# Autodesk Inventor assembly: NX3224T024_011_Ass
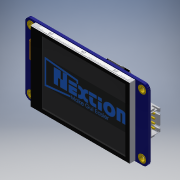
[picture p0: Inventor's stored thumbnail of the model, 180x180]
Saved by Autodesk Inventor 2017 SP1 (Build 210196100, 196)
## iProperties
Created: 2016-08-28
Part Number: NX3224T024_011_Ass
Document SubType Name: Assembly
Designer: jwrjc
Author: jwrjc
## Documents named in this file (14)
- D:\My Projects\Inventor\ElectricalComponents\Nextion_NX3224T024_011\NX3224T024_011_Ass.iam
- D:\My Projects\Inventor\ElectricalComponents\Nextion_NX3224T024_011\NX3224T024_011_PCB.ipt
- D:\My Projects\Inventor\ElectricalComponents\Nextion_NX3224T024_011\AMS1117.ipt
- D:\Documents\Inventor\Content Center Files\R2017\en-US\603_SMD\603_Cap-Lead.ipt
- D:\Documents\Inventor\Content Center Files\R2017\en-US\1206_SMD\1206_Cap.ipt
- D:\My Projects\Inventor\ElectricalComponents\Nextion_NX3224T024_011\603_Resistor.ipt
- D:\My Projects\Inventor\ElectricalComponents\Nextion_NX3224T024_011\IcNextion.ipt
- D:\My Projects\Inventor\ElectricalComponents\Nextion_NX3224T024_011\24_pin_IC.ipt
- D:\My Projects\Inventor\ElectricalComponents\Nextion_NX3224T024_011\16_pin_IC.ipt
- D:\My Projects\Inventor\ElectricalComponents\Nextion_NX3224T024_011\SMD_Trans.ipt
- D:\My Projects\Inventor\ElectricalComponents\Nextion_NX3224T024_011\Micro_SD_Slot.ipt
- D:\My Projects\Inventor\ElectricalComponents\Nextion_NX3224T024_011\SD_Center.ipt
- D:\My Projects\Inventor\ElectricalComponents\Nextion_NX3224T024_011\Nextion_Plug.ipt
- D:\My Projects\Inventor\ElectricalComponents\Nextion_NX3224T024_011\LCD.ipt
## Components (30 placed, 13 different names)
1. NX3224T024_011_PCB:1 — Mate:1, Flush:1, Flush:2, Mate:2, Mate:3, Mate:4, Mate:5, Mate:6, Mate:7, Mate:8, Flush:3, Flush:4, Flush:5, Flush:6, Flush:7, Flush:8, Flush:9, Flush:10, Flush:11, Flush:12, Flush:13, Flush:14, Flush:15, Flush:16, Mate:9, Mate:10, Mate:11, Mate:12, Mate:13, Mate:14, Mate:15, Mate:16, Mate:17, Mate:18, Mate:19, Mate:20, Mate:21, Flush:28, Flush:30, Flush:35, Flush:36, Flush:39, Flush:40, Flush:43, Flush:45, Flush:46, Flush:47, Flush:48, Mate:22, Flush:49, Flush:50
2. AMS1117:1 — Mate:1, Flush:1, Flush:2
3. 603_SMD 603_Cap-Lead:1 — Mate:2, Flush:9, Flush:11
4. 603_SMD 603_Cap-Lead:2 — Mate:3, Flush:8, Flush:10, Flush:37, Flush:38
5. 603_SMD 603_Cap-Lead:3 — Mate:4, Flush:7, Flush:15
6. 603_SMD 603_Cap-Lead:4 — Mate:5, Flush:6, Flush:14, Flush:17, Flush:22
7. 603_SMD 603_Cap-Lead:5 — Mate:6, Flush:5, Flush:12
8. 603_SMD 603_Cap-Lead:6 — Mate:7, Flush:4, Flush:13, Flush:41, Flush:42
9. 1206_SMD 1206_Cap:1 — Mate:8, Flush:3, Flush:16
10. 603_Resistor:1 — Mate:9, Flush:17, Flush:18, Flush:22, Flush:23
11. 603_Resistor:2 — Mate:10, Flush:19, Flush:20, Flush:24, Flush:25
12. 603_Resistor:3 — Mate:11, Flush:21, Flush:26
13. 603_Resistor:4 — Mate:12, Flush:18, Flush:19, Flush:23, Flush:24
14. 603_Resistor:5 — Mate:13, Flush:20, Flush:21, Flush:25, Flush:26
15. 603_Resistor:6 — Mate:14, Flush:27, Flush:29, Flush:36
16. 603_Resistor:7 — Mate:15, Flush:27, Flush:28, Flush:29
17. 603_Resistor:8 — Mate:16, Flush:30, Flush:31, Flush:33
18. 603_Resistor:9 — Mate:17, Flush:31, Flush:32, Flush:33, Flush:34
19. 603_Resistor:10 — Mate:18, Flush:32, Flush:34, Flush:35
20. 603_Resistor:11 — Mate:19, Flush:37, Flush:38
21. 603_Resistor:12 — Mate:20, Flush:41, Flush:42
22. 603_Resistor:13 — Mate:21, Flush:39, Flush:40
23. IcNextion:1
24. 24_pin_IC:1
25. 16_pin_IC:1
26. SMD_Trans:1
27. Micro_SD_Slot:1 — Flush:44, Flush:45
28. SD_Center:1 — Flush:46, Flush:47
29. Nextion_Plug:1 — Flush:48
30. LCD:1 — Mate:22, Flush:49, Flush:50
## Relationships (72: Flush 50, Mate 22)
- Mate:1: NX3224T024_011_PCB:1 ↔ AMS1117:1
- Flush:1 (6 mm): NX3224T024_011_PCB:1 ↔ AMS1117:1
- Flush:2 (12.011 mm): NX3224T024_011_PCB:1 ↔ AMS1117:1
- Mate:2: NX3224T024_011_PCB:1 ↔ 603_SMD 603_Cap-Lead:1
- Mate:3: NX3224T024_011_PCB:1 ↔ 603_SMD 603_Cap-Lead:2
- Mate:4: NX3224T024_011_PCB:1 ↔ 603_SMD 603_Cap-Lead:3
- Mate:5: NX3224T024_011_PCB:1 ↔ 603_SMD 603_Cap-Lead:4
- Mate:6: NX3224T024_011_PCB:1 ↔ 603_SMD 603_Cap-Lead:5
- Mate:7: NX3224T024_011_PCB:1 ↔ 603_SMD 603_Cap-Lead:6
- Mate:8: NX3224T024_011_PCB:1 ↔ 1206_SMD 1206_Cap:1
- Flush:3 (3.4 mm): NX3224T024_011_PCB:1 ↔ 1206_SMD 1206_Cap:1
- Flush:4 (10.345 mm): NX3224T024_011_PCB:1 ↔ 603_SMD 603_Cap-Lead:6
- Flush:5 (6.888 mm): NX3224T024_011_PCB:1 ↔ 603_SMD 603_Cap-Lead:5
- Flush:6 (24.2 mm): NX3224T024_011_PCB:1 ↔ 603_SMD 603_Cap-Lead:4
- Flush:7 (24.4 mm): NX3224T024_011_PCB:1 ↔ 603_SMD 603_Cap-Lead:3
- Flush:8 (21.3 mm): NX3224T024_011_PCB:1 ↔ 603_SMD 603_Cap-Lead:2
- Flush:9 (13 mm): NX3224T024_011_PCB:1 ↔ 603_SMD 603_Cap-Lead:1
- Flush:10 (19.42 mm): NX3224T024_011_PCB:1 ↔ 603_SMD 603_Cap-Lead:2
- Flush:11 (21.524 mm): NX3224T024_011_PCB:1 ↔ 603_SMD 603_Cap-Lead:1
- Flush:12 (35.443 mm): NX3224T024_011_PCB:1 ↔ 603_SMD 603_Cap-Lead:5
- Flush:13 (50.165 mm): NX3224T024_011_PCB:1 ↔ 603_SMD 603_Cap-Lead:6
- Flush:14 (15.799 mm): NX3224T024_011_PCB:1 ↔ 603_SMD 603_Cap-Lead:4
- Flush:15 (29.568 mm): NX3224T024_011_PCB:1 ↔ 603_SMD 603_Cap-Lead:3
- Flush:16 (8.742 mm): NX3224T024_011_PCB:1 ↔ 1206_SMD 1206_Cap:1
- Mate:9: NX3224T024_011_PCB:1 ↔ 603_Resistor:1
- Mate:10: NX3224T024_011_PCB:1 ↔ 603_Resistor:2
- Mate:11: NX3224T024_011_PCB:1 ↔ 603_Resistor:3
- Mate:12: NX3224T024_011_PCB:1 ↔ 603_Resistor:4
- Mate:13: NX3224T024_011_PCB:1 ↔ 603_Resistor:5
- Mate:14: NX3224T024_011_PCB:1 ↔ 603_Resistor:6
- Mate:15: NX3224T024_011_PCB:1 ↔ 603_Resistor:7
- Mate:16: NX3224T024_011_PCB:1 ↔ 603_Resistor:8
- Mate:17: NX3224T024_011_PCB:1 ↔ 603_Resistor:9
- Mate:18: NX3224T024_011_PCB:1 ↔ 603_Resistor:10
- Mate:19: NX3224T024_011_PCB:1 ↔ 603_Resistor:11
- Mate:20: NX3224T024_011_PCB:1 ↔ 603_Resistor:12
- Mate:21: NX3224T024_011_PCB:1 ↔ 603_Resistor:13
- Flush:17 (-0.081 mm): 603_SMD 603_Cap-Lead:4 ↔ 603_Resistor:1
- Flush:18 (-0.002 mm): 603_Resistor:1 ↔ 603_Resistor:4
- Flush:19 (-0.072 mm): 603_Resistor:2 ↔ 603_Resistor:4
- Flush:20 (0.065 mm): 603_Resistor:2 ↔ 603_Resistor:5
- Flush:21 (0.039 mm): 603_Resistor:3 ↔ 603_Resistor:5
- Flush:22 (2.237 mm): 603_SMD 603_Cap-Lead:4 ↔ 603_Resistor:1
- Flush:23 (2.347 mm): 603_Resistor:1 ↔ 603_Resistor:4
- Flush:24 (2.335 mm): 603_Resistor:2 ↔ 603_Resistor:4
- Flush:25 (2.095 mm): 603_Resistor:2 ↔ 603_Resistor:5
- Flush:26 (2.364 mm): 603_Resistor:3 ↔ 603_Resistor:5
- Flush:27 (2.373 mm): 603_Resistor:6 ↔ 603_Resistor:7
- Flush:28 (13.54 mm): NX3224T024_011_PCB:1 ↔ 603_Resistor:7
- Flush:29 (-0.04 mm): 603_Resistor:6 ↔ 603_Resistor:7
- Flush:30 (10.991 mm): NX3224T024_011_PCB:1 ↔ 603_Resistor:8
- Flush:31 (-0.029 mm): 603_Resistor:8 ↔ 603_Resistor:9
- Flush:32 (-0.005 mm): 603_Resistor:9 ↔ 603_Resistor:10
- Flush:33 (2.195 mm): 603_Resistor:8 ↔ 603_Resistor:9
- Flush:34 (2.34 mm): 603_Resistor:9 ↔ 603_Resistor:10
- Flush:35 (19.485 mm): NX3224T024_011_PCB:1 ↔ 603_Resistor:10
- Flush:36 (31.081 mm): NX3224T024_011_PCB:1 ↔ 603_Resistor:6
- Flush:37 (0.013 mm): 603_SMD 603_Cap-Lead:2 ↔ 603_Resistor:11
- Flush:38 (2.394 mm): 603_SMD 603_Cap-Lead:2 ↔ 603_Resistor:11
- Flush:39 (12.49 mm): NX3224T024_011_PCB:1 ↔ 603_Resistor:13
- Flush:40 (7.157 mm): NX3224T024_011_PCB:1 ↔ 603_Resistor:13
- Flush:41 (2.27 mm): 603_SMD 603_Cap-Lead:6 ↔ 603_Resistor:12
- Flush:42 (0.001 mm): 603_SMD 603_Cap-Lead:6 ↔ 603_Resistor:12
- Flush:43 (2 mm): NX3224T024_011_PCB:1
- Flush:44: Micro_SD_Slot:1
- Flush:45: NX3224T024_011_PCB:1 ↔ Micro_SD_Slot:1
- Flush:46: NX3224T024_011_PCB:1 ↔ SD_Center:1
- Flush:47: NX3224T024_011_PCB:1 ↔ SD_Center:1
- Flush:48: NX3224T024_011_PCB:1 ↔ Nextion_Plug:1
- Mate:22: NX3224T024_011_PCB:1 ↔ LCD:1
- Flush:49 (7.7 mm): NX3224T024_011_PCB:1 ↔ LCD:1
- Flush:50 (0.35 mm): NX3224T024_011_PCB:1 ↔ LCD:1
